# Autodesk Inventor assembly: 42146-29
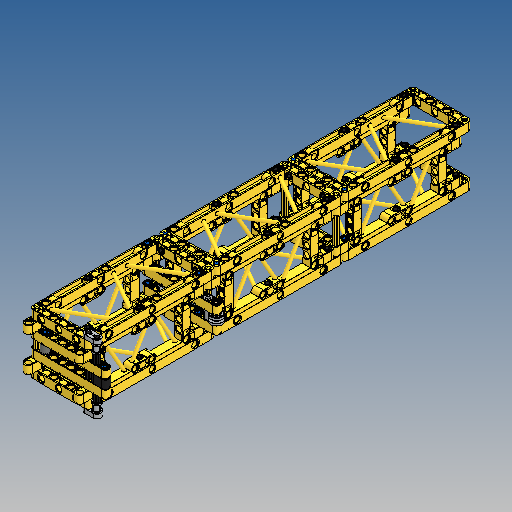
[picture p0: Inventor's stored thumbnail of the model, 512x512]
Saved by Autodesk Inventor 2025 (Build 290162010, 162A)
## iProperties
Created: 2024-12-04
Part Number: 42146-29
Material: Generisch
Document SubType Name: Assembly
Designer: hp.muther
Author: hp.muther
## Documents named in this file (17)
- D:\Inventor\Projekte\Muther\LEGO Technic\LEGO Technik - Raupenkran LR 13000 (42146)\42146-29.iam
- D:\Inventor\Projekte\Muther\LEGO Technic\LEGO Pieces\Rahmen, T-Stücke\79766-Yellow.ipt
- D:\Inventor\Projekte\Muther\LEGO Technic\LEGO Pieces\Pin's\43093-Blue.ipt
- D:\Inventor\Projekte\Muther\LEGO Technic\LEGO Pieces\Pin's\2780-Black.ipt
- D:\Inventor\Projekte\Muther\LEGO Technic\LEGO Pieces\Rahmen, T-Stücke\79767-Yellow.ipt
- D:\Inventor\Projekte\Muther\LEGO Technic\LEGO Pieces\Achsen\44294-Yellow.ipt
- D:\Inventor\Projekte\Muther\LEGO Technic\LEGO Pieces\Pin's\32556-Tan.ipt
- D:\Inventor\Projekte\Muther\LEGO Technic\LEGO Pieces\Räder, Raupe\42610-LtBluishGray.ipt
- D:\Inventor\Projekte\Muther\LEGO Technic\LEGO Pieces\Pin's\77765-MediumStoneGrey.ipt
- D:\Inventor\Projekte\Muther\LEGO Technic\LEGO Pieces\Lochbalken\40490-Yellow.ipt
- D:\Inventor\Projekte\Muther\LEGO Technic\LEGO Pieces\Verbindungselemente\48989-LtBluishGray.ipt
- D:\Inventor\Projekte\Muther\LEGO Technic\LEGO Pieces\Pin's\6558-Blue.ipt
- D:\Inventor\Projekte\Muther\LEGO Technic\LEGO Pieces\Rund\18654-DkBluishGray.ipt
- D:\Inventor\Projekte\Muther\LEGO Technic\LEGO Pieces\Lochbalken\60483-Black.ipt
- D:\Inventor\Projekte\Muther\LEGO Technic\LEGO Pieces\Achsen\3707-Black.ipt
- D:\Inventor\Projekte\Muther\LEGO Technic\LEGO Pieces\Rund\3713-LtBluishGray.ipt
- D:\Inventor\Projekte\Muther\LEGO Technic\LEGO Pieces\Lochbalken schmal\41677-LtBluishGray.ipt
## Components (75 placed, 16 different names)
1. 79766-Yellow:1 — Einfügen:2, Einfügen:3, Einfügen:4, Einfügen:5, Einfügen:6, Einfügen:7, Einfügen:8, Einfügen:9, Einfügen:18, Einfügen:28
2. 43093-Blue:1 — Einfügen:8
3. 43093-Blue:2 — Einfügen:9
4. 2780-Black:1 — Einfügen:2
5. 2780-Black:2 — Einfügen:3
6. 2780-Black:3 — Einfügen:4, Passend:1
7. 2780-Black:4 — Einfügen:5, Passend:3
8. 2780-Black:5 — Einfügen:6
9. 2780-Black:6 — Einfügen:7
10. 79767-Yellow:1 — Einfügen:18, Passend:1
11. 79766-Yellow:2 — Einfügen:10, Einfügen:11, Einfügen:12, Einfügen:13, Einfügen:14, Einfügen:15, Einfügen:16, Einfügen:17, Einfügen:29, Einfügen:39
12. 43093-Blue:3 — Einfügen:10
13. 43093-Blue:4 — Einfügen:11
14. 2780-Black:7 — Einfügen:12
15. 2780-Black:8 — Einfügen:13
16. 2780-Black:9 — Einfügen:14, Passend:6
17. 2780-Black:10 — Einfügen:15, Passend:4
18. 2780-Black:11 — Einfügen:16
19. 2780-Black:12 — Einfügen:17
20. 79767-Yellow:2 — Einfügen:29, Passend:4
21. 79766-Yellow:3 — Einfügen:40
22. 43093-Blue:5
23. 43093-Blue:6
24. 2780-Black:13 — Passend:7
25. 2780-Black:14
26. 2780-Black:15
27. 2780-Black:16
28. 2780-Black:17
29. 2780-Black:18
30. 79767-Yellow:3 — Einfügen:28, Passend:3
31. 79766-Yellow:4 — Einfügen:30, Einfügen:31, Einfügen:32, Einfügen:33, Einfügen:34, Einfügen:35, Einfügen:36, Einfügen:37, Einfügen:38, Einfügen:40, Passend:7, Einfügen:41, Einfügen:42, Einfügen:68
32. 43093-Blue:7 — Einfügen:36
33. 43093-Blue:8 — Einfügen:37
34. 2780-Black:19 — Einfügen:30, Passend:19
35. 2780-Black:20 — Einfügen:31
36. 2780-Black:21 — Einfügen:32
37. 2780-Black:22 — Einfügen:33
38. 2780-Black:23 — Einfügen:34
39. 2780-Black:24 — Einfügen:35
40. 79767-Yellow:4 — Einfügen:38, Einfügen:39, Passend:6
41. 44294-Yellow:1 — Einfügen:41
42. 44294-Yellow:2 — Einfügen:42
43. 32556-Tan:1 — Einfügen:43
44. 42610-LtBluishGray:1 — Einfügen:45
45. 77765-MediumStoneGrey:1 — Einfügen:44
46. 40490-Yellow:1 — Einfügen:43, Einfügen:44, Einfügen:45, Einfügen:46, Passend:8
47. 40490-Yellow:2 — Einfügen:47, Passend:9, Einfügen:52, Passend:13
48. 48989-LtBluishGray:1 — Einfügen:46, Passend:8, Einfügen:47, Passend:9
49. 79767-Yellow:5 — Einfügen:48, Einfügen:49, Einfügen:50, Einfügen:51, Einfügen:52, Einfügen:53, Einfügen:59, Passend:17
50. 2780-Black:25 — Einfügen:51, Passend:10
51. 2780-Black:26 — Einfügen:50
52. 6558-Blue:1 — Einfügen:49
53. 6558-Blue:2 — Einfügen:48
54. 79766-Yellow:5 — Einfügen:53, Passend:10, Passend:12, Einfügen:65, Einfügen:66, Einfügen:69, Einfügen:70
55. 79767-Yellow:6
56. 2780-Black:27
57. 2780-Black:28 — Passend:12
58. 6558-Blue:3
59. 6558-Blue:4 — Passend:13
60. 79766-Yellow:6 — Einfügen:59, Einfügen:68, Passend:19
61. 40490-Yellow:3 — Einfügen:64, Passend:14, Passend:15, Passend:16, Passend:17, Einfügen:71
62. 40490-Yellow:4 — Einfügen:60, Einfügen:61, Einfügen:62, Einfügen:63, Passend:18, Einfügen:72
63. 6558-Blue:5 — Einfügen:60
64. 6558-Blue:6 — Einfügen:61, Passend:14
65. 18654-DkBluishGray:1 — Einfügen:62
66. 60483-Black:1 — Einfügen:63, Einfügen:64, Passend:15, Einfügen:67
67. 44294-Yellow:3 — Einfügen:65, Passend:16
68. 3707-Black:1 — Einfügen:67
69. 3707-Black:2 — Einfügen:66, Passend:18, Passend:21, Passend:22
70. 44294-Yellow:4 — Einfügen:69
71. 44294-Yellow:5 — Einfügen:70
72. 3713-LtBluishGray:1 — Einfügen:71, Einfügen:75
73. 3713-LtBluishGray:2 — Einfügen:72, Einfügen:76
74. 41677-LtBluishGray:1 — Einfügen:75, Passend:22
75. 41677-LtBluishGray:2 — Einfügen:76, Passend:21
## Relationships (94: Insert 73, Mate 21)
- Einfügen:2 [Insert]: 79766-Yellow:1 ↔ 2780-Black:1
- Einfügen:3 [Insert]: 79766-Yellow:1 ↔ 2780-Black:2
- Einfügen:4 [Insert]: 79766-Yellow:1 ↔ 2780-Black:3
- Einfügen:5 [Insert]: 79766-Yellow:1 ↔ 2780-Black:4
- Einfügen:6 [Insert]: 79766-Yellow:1 ↔ 2780-Black:5
- Einfügen:7 [Insert]: 79766-Yellow:1 ↔ 2780-Black:6
- Einfügen:8 [Insert]: 79766-Yellow:1 ↔ 43093-Blue:1
- Einfügen:9 [Insert]: 79766-Yellow:1 ↔ 43093-Blue:2
- Einfügen:10 [Insert]: 79766-Yellow:2 ↔ 43093-Blue:3
- Einfügen:11 [Insert]: 79766-Yellow:2 ↔ 43093-Blue:4
- Einfügen:12 [Insert]: 79766-Yellow:2 ↔ 2780-Black:7
- Einfügen:13 [Insert]: 79766-Yellow:2 ↔ 2780-Black:8
- Einfügen:14 [Insert]: 79766-Yellow:2 ↔ 2780-Black:9
- Einfügen:15 [Insert]: 79766-Yellow:2 ↔ 2780-Black:10
- Einfügen:16 [Insert]: 79766-Yellow:2 ↔ 2780-Black:11
- Einfügen:17 [Insert]: 79766-Yellow:2 ↔ 2780-Black:12
- Einfügen:18 [Insert]: 79766-Yellow:1 ↔ 79767-Yellow:1
- Passend:1 [Mate]: 2780-Black:3 ↔ 79767-Yellow:1
- [Insert]: 79766-Yellow:3 ↔ 2780-Black:13
- [Insert]: 79766-Yellow:3 ↔ 2780-Black:14
- [Insert]: 79766-Yellow:3 ↔ 2780-Black:15
- [Insert]: 79766-Yellow:3 ↔ 2780-Black:16
- [Insert]: 79766-Yellow:3 ↔ 2780-Black:17
- [Insert]: 79766-Yellow:3 ↔ 2780-Black:18
- [Insert]: 79766-Yellow:3 ↔ 43093-Blue:5
- [Insert]: 79766-Yellow:3 ↔ 43093-Blue:6
- [Insert]: 79766-Yellow:3 ↔ 79767-Yellow:3
- [Mate]: 2780-Black:15 ↔ 79767-Yellow:3
- Einfügen:28 [Insert]: 79766-Yellow:1 ↔ 79767-Yellow:3
- Passend:3 [Mate]: 2780-Black:4 ↔ 79767-Yellow:3
- Einfügen:29 [Insert]: 79766-Yellow:2 ↔ 79767-Yellow:2
- Passend:4 [Mate]: 2780-Black:10 ↔ 79767-Yellow:2
- Einfügen:30 [Insert]: 79766-Yellow:4 ↔ 2780-Black:19
- Einfügen:31 [Insert]: 79766-Yellow:4 ↔ 2780-Black:20
- Einfügen:32 [Insert]: 79766-Yellow:4 ↔ 2780-Black:21
- Einfügen:33 [Insert]: 79766-Yellow:4 ↔ 2780-Black:22
- Einfügen:34 [Insert]: 79766-Yellow:4 ↔ 2780-Black:23
- Einfügen:35 [Insert]: 79766-Yellow:4 ↔ 2780-Black:24
- Einfügen:36 [Insert]: 79766-Yellow:4 ↔ 43093-Blue:7
- Einfügen:37 [Insert]: 79766-Yellow:4 ↔ 43093-Blue:8
- Einfügen:38 [Insert]: 79766-Yellow:4 ↔ 79767-Yellow:4
- [Mate]: 2780-Black:21 ↔ 79767-Yellow:4
- Einfügen:39 [Insert]: 79766-Yellow:2 ↔ 79767-Yellow:4
- Passend:6 [Mate]: 2780-Black:9 ↔ 79767-Yellow:4
- Einfügen:40 [Insert]: 79766-Yellow:3 ↔ 79766-Yellow:4
- Passend:7 [Mate]: 2780-Black:13 ↔ 79766-Yellow:4
- Einfügen:41 [Insert]: 79766-Yellow:4 ↔ 44294-Yellow:1
- Einfügen:42 [Insert]: 79766-Yellow:4 ↔ 44294-Yellow:2
- Einfügen:43 [Insert]: 32556-Tan:1 ↔ 40490-Yellow:1
- Einfügen:44 [Insert]: 77765-MediumStoneGrey:1 ↔ 40490-Yellow:1
- Einfügen:45 [Insert]: 42610-LtBluishGray:1 ↔ 40490-Yellow:1
- Einfügen:46 [Insert]: 40490-Yellow:1 ↔ 48989-LtBluishGray:1
- Passend:8 [Mate]: 40490-Yellow:1 ↔ 48989-LtBluishGray:1
- Einfügen:47 [Insert]: 40490-Yellow:2 ↔ 48989-LtBluishGray:1
- Passend:9 [Mate]: 40490-Yellow:2 ↔ 48989-LtBluishGray:1
- Einfügen:48 [Insert]: 79767-Yellow:5 ↔ 6558-Blue:2
- Einfügen:49 [Insert]: 79767-Yellow:5 ↔ 6558-Blue:1
- Einfügen:50 [Insert]: 79767-Yellow:5 ↔ 2780-Black:26
- Einfügen:51 [Insert]: 79767-Yellow:5 ↔ 2780-Black:25
- Einfügen:52 [Insert] (0.8 mm): 40490-Yellow:2 ↔ 79767-Yellow:5
- Einfügen:53 [Insert]: 79767-Yellow:5 ↔ 79766-Yellow:5
- Passend:10 [Mate]: 2780-Black:25 ↔ 79766-Yellow:5
- [Insert]: 79767-Yellow:6 ↔ 6558-Blue:4
- [Insert]: 79767-Yellow:6 ↔ 6558-Blue:3
- [Insert]: 79767-Yellow:6 ↔ 2780-Black:28
- [Insert]: 79767-Yellow:6 ↔ 2780-Black:27
- [Insert]: 79767-Yellow:6 ↔ 79766-Yellow:6
- [Mate]: 2780-Black:27 ↔ 79766-Yellow:6
- Einfügen:59 [Insert]: 79767-Yellow:5 ↔ 79766-Yellow:6
- Passend:12 [Mate]: 79766-Yellow:5 ↔ 2780-Black:28
- Passend:13 [Mate]: 40490-Yellow:2 ↔ 6558-Blue:4
- Einfügen:60 [Insert]: 40490-Yellow:4 ↔ 6558-Blue:5
- Einfügen:61 [Insert]: 40490-Yellow:4 ↔ 6558-Blue:6
- Einfügen:62 [Insert]: 40490-Yellow:4 ↔ 18654-DkBluishGray:1
- Einfügen:63 [Insert]: 40490-Yellow:4 ↔ 60483-Black:1
- Einfügen:64 [Insert]: 40490-Yellow:3 ↔ 60483-Black:1
- Passend:14 [Mate]: 40490-Yellow:3 ↔ 6558-Blue:6
- Passend:15 [Mate]: 40490-Yellow:3 ↔ 60483-Black:1
- Einfügen:65 [Insert]: 79766-Yellow:5 ↔ 44294-Yellow:3
- Passend:16 [Mate]: 40490-Yellow:3 ↔ 44294-Yellow:3
- Passend:17 [Mate]: 79767-Yellow:5 ↔ 40490-Yellow:3
- Einfügen:66 [Insert] (-60 mm): 79766-Yellow:5 ↔ 3707-Black:2
- Einfügen:67 [Insert] (-36 mm): 60483-Black:1 ↔ 3707-Black:1
- Einfügen:68 [Insert]: 79766-Yellow:4 ↔ 79766-Yellow:6
- Passend:18 [Mate]: 40490-Yellow:4 ↔ 3707-Black:2
- Passend:19 [Mate]: 2780-Black:19 ↔ 79766-Yellow:6
- Einfügen:69 [Insert]: 79766-Yellow:5 ↔ 44294-Yellow:4
- Einfügen:70 [Insert]: 79766-Yellow:5 ↔ 44294-Yellow:5
- Einfügen:71 [Insert] (8 mm): 40490-Yellow:3 ↔ 3713-LtBluishGray:1
- Einfügen:72 [Insert] (8 mm): 40490-Yellow:4 ↔ 3713-LtBluishGray:2
- Einfügen:75 [Insert]: 3713-LtBluishGray:1 ↔ 41677-LtBluishGray:1
- Einfügen:76 [Insert]: 3713-LtBluishGray:2 ↔ 41677-LtBluishGray:2
- Passend:21 [Mate]: 3707-Black:2 ↔ 41677-LtBluishGray:2
- Passend:22 [Mate]: 3707-Black:2 ↔ 41677-LtBluishGray:1
## Named parameters: d18_d16 = 0 mm, d19_d17 = 0 mm, d20_d1 = 0 mm, d21_d2 = 0 mm, d22_d3 = 0 mm, d23_d4 = 0 mm, d24_d5 = 0 mm, d25_d6 = 0 mm, d26_d7 = 0 mm, d27_d0 = 0 mm, d32_d16 = 0 mm, d33_d17 = 0 mm, d34_d1 = 0 mm, d35_d2 = 0 mm, d36_d3 = 0 mm, d37_d4 = 0 mm, d38_d5 = 0 mm, d39_d6 = 0 mm, d40_d7 = 0 mm, d41_d0 = 0 mm, d62_d55 = 0 mm, d63_d56 = 0 mm, d64_d57 = 0 mm, d65_d58 = 0 mm, d66_d60 = 0 mm, d67_d61 = 0 mm
